# Autodesk Inventor assembly: Walking Leg Test
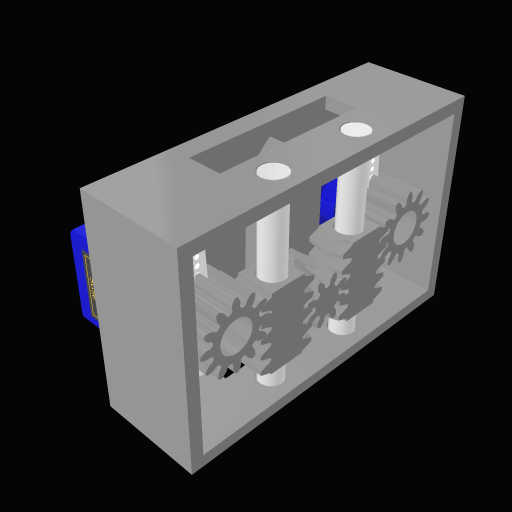
[picture p0: Inventor's stored thumbnail of the model, 512x512]
Saved by Autodesk Inventor 2023.2 (Build 272271030, 271C)
## iProperties
Created: 2023-10-23
Part Number: Walking Leg Test
Document SubType Name: Assembly
Designer: robpl
Author: robpl
## Documents named in this file (7)
- C:\Users\robpl\OneDrive\Documents\Inventor\Battlebots\Walking Leg Test.iam
- C:\Users\robpl\OneDrive\Documents\Inventor\Battlebots\Walking Test\SG90 - Micro Servo 9g - Tower Pro\SG90 - Micro Servo 9g - Tower Pro.ipt
- C:\Users\robpl\OneDrive\Documents\Inventor\Battlebots\Walking Test\rack.ipt
- C:\Users\robpl\OneDrive\Documents\Inventor\Battlebots\Walking Test\gear.ipt
- C:\Users\robpl\OneDrive\Documents\Inventor\Battlebots\Walking Test\Rack and Pinion Test\Test Frame.ipt
- C:\Users\robpl\OneDrive\Documents\Inventor\Battlebots\Walking Leg Test\Servo Gear.ipt
- C:\Users\robpl\OneDrive\Documents\Inventor\Battlebots\Walking Leg Test\Rail.ipt
## Components (10 placed, 6 different names)
1. SG90 - Micro Servo 9g - Tower Pro:2 — Mate:6, Mate:7, Mate:8, Mate:9, Mate:10, Angle:1
2. rack:1 — Flush:1, Mate:1, Flush:2, Flush:3, Mate:5, Mate:11, Flush:4, Angle:2
3. gear:1 — Flush:1, Mate:1, Mate:5
4. rack:2 — Flush:2, Flush:3, Mate:17
5. Test Frame:1 — Mate:6, Mate:7, Mate:8, Angle:2, Mate:12, Mate:13, Mate:14, Mate:17, Mate:18, Mate:19, Flush:5, Flush:6
6. Servo Gear:1 — Mate:9, Mate:10, Angle:1, Mate:11, Flush:4
7. SG90 - Micro Servo 9g - Tower Pro:3 — Mate:12, Mate:13, Mate:14, Mate:15, Mate:16
8. Servo Gear:2 — Mate:15, Mate:16
9. Rail:1 — Mate:18, Flush:5
10. Rail:2 — Mate:19, Flush:6
## Relationships (24: Mate 16, Flush 6, Angle 2)
- Flush:1 (-0.5 mm): rack:1 ↔ gear:1
- Mate:1 (5 mm): rack:1 ↔ gear:1
- Flush:2: rack:1 ↔ rack:2
- Flush:3: rack:1 ↔ rack:2
- Mate:5 (-10 mm): rack:1 ↔ gear:1
- Mate:6: SG90 - Micro Servo 9g - Tower Pro:2 ↔ Test Frame:1
- Mate:7: SG90 - Micro Servo 9g - Tower Pro:2 ↔ Test Frame:1
- Mate:8: SG90 - Micro Servo 9g - Tower Pro:2 ↔ Test Frame:1
- Mate:9: SG90 - Micro Servo 9g - Tower Pro:2 ↔ Servo Gear:1
- Mate:10: SG90 - Micro Servo 9g - Tower Pro:2 ↔ Servo Gear:1
- Angle:1 (15 deg): SG90 - Micro Servo 9g - Tower Pro:2 ↔ Servo Gear:1
- Mate:11 (7.5 mm): rack:1 ↔ Servo Gear:1
- Flush:4: rack:1 ↔ Servo Gear:1
- Angle:2 (0 deg): rack:1 ↔ Test Frame:1
- Mate:12: Test Frame:1 ↔ SG90 - Micro Servo 9g - Tower Pro:3
- Mate:13: Test Frame:1 ↔ SG90 - Micro Servo 9g - Tower Pro:3
- Mate:14: Test Frame:1 ↔ SG90 - Micro Servo 9g - Tower Pro:3
- Mate:15: SG90 - Micro Servo 9g - Tower Pro:3 ↔ Servo Gear:2
- Mate:16: SG90 - Micro Servo 9g - Tower Pro:3 ↔ Servo Gear:2
- Mate:17: rack:2 ↔ Test Frame:1
- Mate:18: Test Frame:1 ↔ Rail:1
- Mate:19: Test Frame:1 ↔ Rail:2
- Flush:5: Test Frame:1 ↔ Rail:1
- Flush:6: Test Frame:1 ↔ Rail:2
